# Autodesk Inventor assembly: Body Assembly
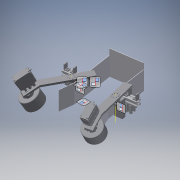
[picture p0: Inventor's stored thumbnail of the model, 180x180]
Saved by Autodesk Inventor 2019 (Build 230136000, 136)
## iProperties
Created: 2019-10-15
Part Number: Body Assembly
Document SubType Name: Assembly
Designer: User
Author: User
## Documents named in this file (24)
- C:\Robotics\2019-20_CAD\Collection\Body Assembly.iam
- C:\Robotics\2019-20_CAD\Collection\U-Part Gen 2.ipt
- C:\Robotics\COTSParts\Actobotics\545 parts\545364 assembly.ipt
- C:\Robotics\2019-20_CAD\Collection\wheel arm stand off.ipt
- C:\Robotics\2019-20_CAD\Collection\arm assembaly.iam
- C:\Robotics\COTSParts\Vex\2-Wire_Motor_393_276-2177.iam
- C:\Robotics\COTSParts\Wheels\2.5inFoamWheel250TMD.ipt
- C:\Robotics\2019-20_CAD\Collection\vex motor adaptor to tetrix.ipt
- C:\Robotics\COTSParts\Bearings - AndyMark\Bearing 250 ID 500 OD flanged.ipt
- C:\Robotics\COTSParts\Bosch Extrusion\Bosch 20x20 - 1.5 Part.Shoot.ipt
- C:\Robotics\COTSParts\Bosch Extrusion\Bosch 20x20 - 4.5 Part.Shoot.ipt
- C:\Robotics\2019-20_CAD\Collection\spring tab for on 20x20.ipt
- C:\Robotics\2019-20_CAD\Collection\stop for on 20x20.ipt
- C:\Robotics\COTSParts\Actobotics\545 parts\545364 assembly_MIR.ipt
- C:\Robotics\2019-20_CAD\Collection\wheel arm stand off_MIR.ipt
- C:\Robotics\2019-20_CAD\Collection\arm assembaly_MIR.iam
- C:\Robotics\COTSParts\Vex\2-Wire_Motor_393_276-2177_MIR.iam
- C:\Robotics\2019-20_CAD\Collection\vex motor adaptor to tetrix_MIR.ipt
- C:\Robotics\COTSParts\Wheels\2.5inFoamWheel250TMD_MIR.ipt
- C:\Robotics\COTSParts\Bearings - AndyMark\Bearing 250 ID 500 OD flanged_MIR1.ipt
- C:\Robotics\COTSParts\Bosch Extrusion\Bosch 20x20 - 1.5 Part.Shoot_MIR.ipt
- C:\Robotics\COTSParts\Bosch Extrusion\Bosch 20x20 - 4.5 Part.Shoot_MIR.ipt
- C:\Robotics\2019-20_CAD\Collection\spring tab for on 20x20_MIR.ipt
- C:\Robotics\2019-20_CAD\Collection\stop for on 20x20_MIR.ipt
## Components (23 placed, 22 different names)
1. U-Part Gen 2:1 — Mate:23, Flush:10, Mate:36, Mate:40, Flush:24, Flush:25, Flush:26, Flush:27, Mate:57
2. 545364 assembly:2 — Mate:17, Mate:18, Mate:20
3. wheel arm stand off:2 — Mate:17, Mate:18, Mate:22, Mate:23, Flush:10, Mate:38, Flush:25, Flush:28
4. arm assembaly:1 [sub-assembly] — Mate:20, Mate:22, Mate:24, Mate:25, Mate:26, Mate:28, Mate:32
5. 2-Wire_Motor_393_276-2177:1 [sub-assembly] — Mate:24, Mate:25, Mate:26, Mate:27
6. vex motor adaptor to tetrix:1 — Mate:27, Mate:28, Mate:29, Insert:1, Mate:30, Mate:31
7. 2.5inFoamWheel250TMD:1 — Mate:29, Insert:1, Mate:30
8. Bearing 250 ID 500 OD flanged:1 — Mate:31, Mate:32
9. Bosch 20x20 - 1.5 Part.Shoot:2 — Mate:35, Flush:12, Flush:13, Mate:38, Flush:24
10. Bosch 20x20 - 4.5 Part.Shoot:1 — Mate:35, Flush:12, Mate:36, Flush:13, Mate:39, Flush:14, Flush:16
11. spring tab for on arm:1 — Mate:39, Mate:40, Flush:14, Flush:15, Flush:17
12. spring tab for on arm:2 — Flush:15, Flush:16, Flush:17
13. 545364 assembly_MIR:1 — Mate:41, Mate:42, Mate:44
14. wheel arm stand off_MIR:1 — Mate:41, Mate:42, Mate:43, Mate:54, Flush:27, Mate:57, Flush:28
15. arm assembaly_MIR:1 [sub-assembly] — Mate:43, Mate:44, Mate:45, Mate:46, Mate:47, Mate:48, Mate:52
16. 2-Wire_Motor_393_276-2177_MIR:1 [sub-assembly] — Mate:45, Mate:46, Mate:47, Mate:49
17. vex motor adaptor to tetrix_MIR:1 — Mate:48, Mate:49, Mate:50, Insert:2, Mate:51, Mate:53
18. 2.5inFoamWheel250TMD_MIR:1 — Mate:50, Insert:2, Mate:51
19. Bearing 250 ID 500 OD flanged_MIR1:1 — Mate:52, Mate:53
20. Bosch 20x20 - 1.5 Part.Shoot_MIR:1 — Mate:54, Flush:18, Flush:19, Mate:55, Flush:26
21. Bosch 20x20 - 4.5 Part.Shoot_MIR:1 — Flush:18, Flush:19, Mate:55, Flush:20, Mate:56, Flush:22
22. spring tab for on 20x20_MIR:1 — Flush:20, Mate:56, Flush:21, Flush:23
23. stop for on 20x20_MIR:1 — Flush:21, Flush:22, Flush:23
## Relationships (56: Mate 36, Flush 18, Insert 2)
- Mate:17: 545364 assembly:2 ↔ wheel arm stand off:2
- Mate:18: 545364 assembly:2 ↔ wheel arm stand off:2
- Mate:20: 545364 assembly:2 ↔ arm assembaly:1
- Mate:22: wheel arm stand off:2 ↔ arm assembaly:1
- Mate:23 (4.7625 mm): U-Part Gen 2:1 ↔ wheel arm stand off:2
- Flush:10 (-121.1072 mm): U-Part Gen 2:1 ↔ wheel arm stand off:2
- Mate:24: arm assembaly:1 ↔ 2-Wire_Motor_393_276-2177:1
- Mate:25: arm assembaly:1 ↔ 2-Wire_Motor_393_276-2177:1
- Mate:26: arm assembaly:1 ↔ 2-Wire_Motor_393_276-2177:1
- Mate:27: 2-Wire_Motor_393_276-2177:1 ↔ vex motor adaptor to tetrix:1
- Mate:28: arm assembaly:1 ↔ vex motor adaptor to tetrix:1
- Mate:29: vex motor adaptor to tetrix:1 ↔ 2.5inFoamWheel250TMD:1
- Insert:1: vex motor adaptor to tetrix:1 ↔ 2.5inFoamWheel250TMD:1
- Mate:30: vex motor adaptor to tetrix:1 ↔ 2.5inFoamWheel250TMD:1
- Mate:31: vex motor adaptor to tetrix:1 ↔ Bearing 250 ID 500 OD flanged:1
- Mate:32: arm assembaly:1 ↔ Bearing 250 ID 500 OD flanged:1
- Mate:35: Bosch 20x20 - 1.5 Part.Shoot:2 ↔ Bosch 20x20 - 4.5 Part.Shoot:1
- Flush:12: Bosch 20x20 - 1.5 Part.Shoot:2 ↔ Bosch 20x20 - 4.5 Part.Shoot:1
- Mate:36: U-Part Gen 2:1 ↔ Bosch 20x20 - 4.5 Part.Shoot:1
- Flush:13 (15.4051 mm): Bosch 20x20 - 1.5 Part.Shoot:2 ↔ Bosch 20x20 - 4.5 Part.Shoot:1
- Mate:38 (18.1102 mm): wheel arm stand off:2 ↔ Bosch 20x20 - 1.5 Part.Shoot:2
- Mate:39: Bosch 20x20 - 4.5 Part.Shoot:1 ↔ spring tab for on arm:1
- Mate:40: U-Part Gen 2:1 ↔ spring tab for on arm:1
- Flush:14 (3.65 mm): Bosch 20x20 - 4.5 Part.Shoot:1 ↔ spring tab for on arm:1
- Flush:15: spring tab for on arm:1 ↔ spring tab for on arm:2
- Flush:16: Bosch 20x20 - 4.5 Part.Shoot:1 ↔ spring tab for on arm:2
- Flush:17: spring tab for on arm:1 ↔ spring tab for on arm:2
- Mate:41: 545364 assembly_MIR:1 ↔ wheel arm stand off_MIR:1
- Mate:42: 545364 assembly_MIR:1 ↔ wheel arm stand off_MIR:1
- Mate:43: wheel arm stand off_MIR:1 ↔ arm assembaly_MIR:1
- Mate:44: 545364 assembly_MIR:1 ↔ arm assembaly_MIR:1
- Mate:45: arm assembaly_MIR:1 ↔ 2-Wire_Motor_393_276-2177_MIR:1
- Mate:46: arm assembaly_MIR:1 ↔ 2-Wire_Motor_393_276-2177_MIR:1
- Mate:47: arm assembaly_MIR:1 ↔ 2-Wire_Motor_393_276-2177_MIR:1
- Mate:48: arm assembaly_MIR:1 ↔ vex motor adaptor to tetrix_MIR:1
- Mate:49: 2-Wire_Motor_393_276-2177_MIR:1 ↔ vex motor adaptor to tetrix_MIR:1
- Mate:50: vex motor adaptor to tetrix_MIR:1 ↔ 2.5inFoamWheel250TMD_MIR:1
- Insert:2: vex motor adaptor to tetrix_MIR:1 ↔ 2.5inFoamWheel250TMD_MIR:1
- Mate:51: vex motor adaptor to tetrix_MIR:1 ↔ 2.5inFoamWheel250TMD_MIR:1
- Mate:52: arm assembaly_MIR:1 ↔ Bearing 250 ID 500 OD flanged_MIR1:1
- Mate:53: vex motor adaptor to tetrix_MIR:1 ↔ Bearing 250 ID 500 OD flanged_MIR1:1
- Mate:54 (18.1102 mm): wheel arm stand off_MIR:1 ↔ Bosch 20x20 - 1.5 Part.Shoot_MIR:1
- Flush:18 (15.4051 mm): Bosch 20x20 - 1.5 Part.Shoot_MIR:1 ↔ Bosch 20x20 - 4.5 Part.Shoot_MIR:1
- Flush:19: Bosch 20x20 - 1.5 Part.Shoot_MIR:1 ↔ Bosch 20x20 - 4.5 Part.Shoot_MIR:1
- Mate:55: Bosch 20x20 - 1.5 Part.Shoot_MIR:1 ↔ Bosch 20x20 - 4.5 Part.Shoot_MIR:1
- Flush:20 (3.65 mm): Bosch 20x20 - 4.5 Part.Shoot_MIR:1 ↔ spring tab for on 20x20_MIR:1
- Mate:56: Bosch 20x20 - 4.5 Part.Shoot_MIR:1 ↔ spring tab for on 20x20_MIR:1
- Flush:21: spring tab for on 20x20_MIR:1 ↔ stop for on 20x20_MIR:1
- Flush:22: Bosch 20x20 - 4.5 Part.Shoot_MIR:1 ↔ stop for on 20x20_MIR:1
- Flush:23: spring tab for on 20x20_MIR:1 ↔ stop for on 20x20_MIR:1
- Flush:24: U-Part Gen 2:1 ↔ Bosch 20x20 - 1.5 Part.Shoot:2
- Flush:25: U-Part Gen 2:1 ↔ wheel arm stand off:2
- Flush:26: U-Part Gen 2:1 ↔ Bosch 20x20 - 1.5 Part.Shoot_MIR:1
- Flush:27: U-Part Gen 2:1 ↔ wheel arm stand off_MIR:1
- Mate:57: U-Part Gen 2:1 ↔ wheel arm stand off_MIR:1
- Flush:28: wheel arm stand off:2 ↔ wheel arm stand off_MIR:1
